# Autodesk Inventor assembly: MultiPass0V-OnlyRays
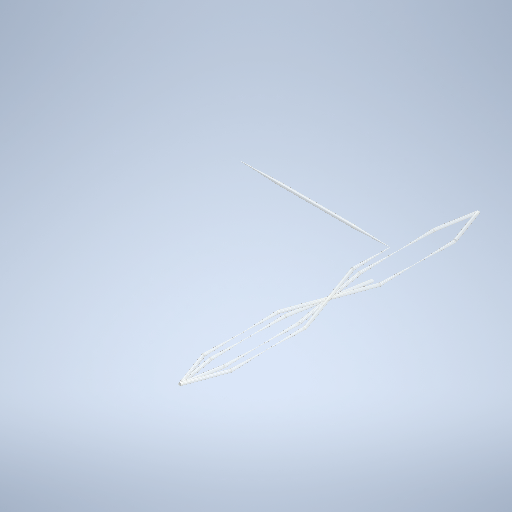
[picture p0: Inventor's stored thumbnail of the model, 512x512]
Saved by Autodesk Inventor 2025 (Build 290162010, 162A)
## iProperties
Created: 2024-08-19
Part Number: MultiPass0V-OnlyRays
Document SubType Name: Assembly
Designer: User
Author: User
## Documents named in this file (7)
- C:\Users\User\Desktop\Hari_Laptop_Contents\KerlinLab\KTN\Multipass\MechanicalDrawing\MultiPass0V-OnlyRays.iam
- C:\Users\User\Desktop\Hari_Laptop_Contents\KerlinLab\KTN\Multipass\MechanicalDrawing\LaserBeamEntry2.ipt
- C:\Users\User\Desktop\Hari_Laptop_Contents\KerlinLab\KTN\Multipass\MechanicalDrawing\LaserBeamCenter1.ipt
- C:\Users\User\Desktop\Hari_Laptop_Contents\KerlinLab\KTN\Multipass\MechanicalDrawing\LaserBeamMirrorAngle1.ipt
- C:\Users\User\Desktop\Hari_Laptop_Contents\KerlinLab\KTN\Multipass\MechanicalDrawing\LaserBeamCenter2.ipt
- C:\Users\User\Desktop\Hari_Laptop_Contents\KerlinLab\KTN\Multipass\MechanicalDrawing\LaserBeamMirrorAngle2.ipt
- C:\Users\User\Desktop\Hari_Laptop_Contents\KerlinLab\KTN\Multipass\MechanicalDrawing\LoopPlane1.ipt
## Components (27 placed, 6 different names)
1. LaserBeamCenter1:1 — Mate:46
2. LaserBeamEntry2:5
3. LaserBeamEntry2:6 — Mate:62
4. LaserBeamEntry2:8
5. LaserBeamEntry2:9
6. LaserBeamEntry2:10
7. LaserBeamCenter1:2 — Mate:58
8. LaserBeamEntry2:11 — Mate:62
9. LaserBeamMirrorAngle1:1 — Mate:67, Mate:101
10. LaserBeamMirrorAngle1:2 — Mate:67
11. LaserBeamMirrorAngle1:3
12. LaserBeamMirrorAngle1:4
13. LaserBeamEntry2:12
14. LaserBeamEntry2:13
15. LaserBeamEntry2:14
16. LaserBeamEntry2:15
17. LaserBeamEntry2:16
18. LaserBeamEntry2:17
19. LaserBeamEntry2:18 — Mate:93
20. LaserBeamCenter2:1 — Mate:91
21. LaserBeamCenter2:2 — Mate:90, Mate:93
22. LaserBeamEntry2:19 — Mate:96, Mate:109
23. LaserBeamMirrorAngle2:1 — Mate:101, Mate:103
24. LaserBeamMirrorAngle2:2 — Mate:103
25. LaserBeamCenter1:3 — Mate:109, Mate:111
26. LaserBeamEntry2:20 — Mate:111
27. LoopPlane1:1 — Mate:113
## Relationships (17: Mate 17)
- Mate:22
- Mate:23
- Mate:24
- Mate:25
- Mate:46: LaserBeamCenter1:1
- Mate:58: LaserBeamCenter1:2
- Mate:62: LaserBeamEntry2:6 ↔ LaserBeamEntry2:11
- Mate:67: LaserBeamMirrorAngle1:1 ↔ LaserBeamMirrorAngle1:2
- Mate:90: LaserBeamCenter2:2
- Mate:91: LaserBeamCenter2:1
- Mate:93 (0.5 mm): LaserBeamEntry2:18 ↔ LaserBeamCenter2:2
- Mate:96: LaserBeamEntry2:19
- Mate:101: LaserBeamMirrorAngle1:1 ↔ LaserBeamMirrorAngle2:1
- Mate:103: LaserBeamMirrorAngle2:1 ↔ LaserBeamMirrorAngle2:2
- Mate:109: LaserBeamEntry2:19 ↔ LaserBeamCenter1:3
- Mate:111: LaserBeamCenter1:3 ↔ LaserBeamEntry2:20
- Mate:113: LoopPlane1:1
